# Autodesk Inventor assembly: Project_Box_Complete_Assembly
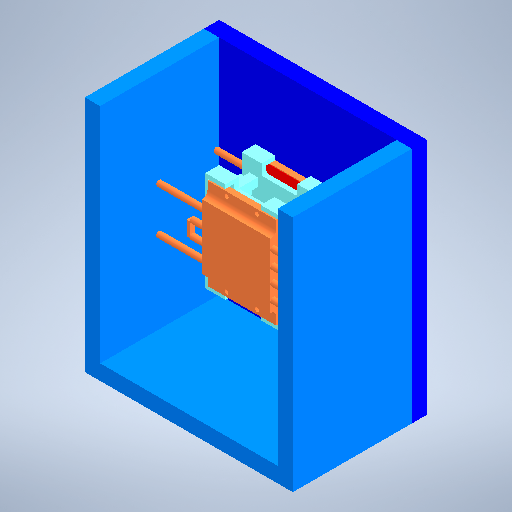
[picture p0: Inventor's stored thumbnail of the model, 512x512]
Saved by Autodesk Inventor 2025.2 (Build 292293000, 293)
## iProperties
Created: 2025-08-10
Part Number: Project_Box_Complete_Assembly
Document SubType Name: Assembly
Designer: cbast
Author: cbast
## Documents named in this file (6)
- C:\Users\cbast\OneDrive\Documents\GitHub\Smart-Pack-for-Advanced-Research-and-Control\variations\Camden\V0.2\Project_Box_Complete_Assembly.iam
- C:\Users\cbast\OneDrive\Documents\GitHub\Smart-Pack-for-Advanced-Research-and-Control\variations\Camden\V0.2\Pillars_18650_Assembly.iam
- C:\Users\cbast\OneDrive\Documents\insul2.ipt
- C:\Users\cbast\OneDrive\Documents\insul3.ipt
- C:\Users\cbast\OneDrive\Documents\GitHub\Smart-Pack-for-Advanced-Research-and-Control\variations\Camden\V0.2\Project Box CAD\RITTAL Enclosure\JB161410HC (1).iam
- C:\Users\cbast\OneDrive\Documents\insulation.ipt
## Components (7 placed, 5 different names)
1. JB161410HC (1):1 [sub-assembly] — Mate:1, Mate:2, Mate:3, Mate:4, Mate:5, Mate:7, Mate:9, Mate:10, Mate:13
2. insulation:1 — Mate:1, Mate:2, Mate:3, Mate:6, Mate:8, Mate:11, Mate:14, Mate:16
3. insul2:1 — Mate:4, Mate:5, Mate:6, Mate:12, Mate:17
4. insul2:2 — Mate:7, Mate:8, Mate:9, Mate:15
5. insul3:2 — Mate:10, Mate:11, Mate:12
6. insul3:3 — Mate:13, Mate:14, Mate:15
7. Pillars_18650_Assembly:1 [sub-assembly] — Mate:16, Mate:17
## Relationships (17: Mate 17)
- Mate:1: JB161410HC (1):1 ↔ insulation:1
- Mate:2: JB161410HC (1):1 ↔ insulation:1
- Mate:3: JB161410HC (1):1 ↔ insulation:1
- Mate:4: JB161410HC (1):1 ↔ insul2:1
- Mate:5: JB161410HC (1):1 ↔ insul2:1
- Mate:6: insulation:1 ↔ insul2:1
- Mate:7: JB161410HC (1):1 ↔ insul2:2
- Mate:8: insulation:1 ↔ insul2:2
- Mate:9: JB161410HC (1):1 ↔ insul2:2
- Mate:10: JB161410HC (1):1 ↔ insul3:2
- Mate:11: insulation:1 ↔ insul3:2
- Mate:12: insul2:1 ↔ insul3:2
- Mate:13: JB161410HC (1):1 ↔ insul3:3
- Mate:14: insulation:1 ↔ insul3:3
- Mate:15: insul2:2 ↔ insul3:3
- Mate:16: insulation:1 ↔ Pillars_18650_Assembly:1
- Mate:17: insul2:1 ↔ Pillars_18650_Assembly:1
